# Autodesk Inventor assembly: RotatingRingAndGear
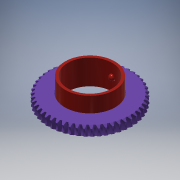
[picture p0: Inventor's stored thumbnail of the model, 180x180]
Saved by Autodesk Inventor 2019.3 (Build 233278000, 278)
## iProperties
Created: 2018-12-30
Part Number: RotatingRingAndGear
Document SubType Name: Assembly
Designer: steele
Author: steele
## Documents named in this file (3)
- C:\git\CAD-Development\robSteele\ShapeWays\TelescopeProjects\Focuser\RotatingRingAndGear.iam
- C:\git\CAD-Development\robSteele\ShapeWays\TelescopeProjects\Focuser\ExternalMotorizedOuterRing.ipt
- C:\git\CAD-Development\robSteele\ShapeWays\TelescopeProjects\Focuser\ExternalMotorizedOuterRingAssembly\Design Accelerator\Worm Gear8.ipt
## Components (2 placed, 2 different names)
1. ExternalMotorizedOuterRing:1 — Insert:1
2. Worm Gear:1 — Insert:1
## Relationships (1: Insert 1)
- Insert:1: ExternalMotorizedOuterRing:1 ↔ Worm Gear:1
